# Autodesk Inventor assembly: Hatch design
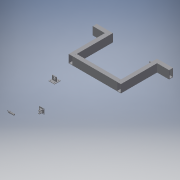
[picture p0: Inventor's stored thumbnail of the model, 180x180]
Saved by Autodesk Inventor 2018 (Build 220112000, 112)
## iProperties
Created: 2019-01-16
Part Number: Hatch design
Document SubType Name: Assembly
Designer: s-4008082
Author: s-4008082
## Documents named in this file (7)
- C:\Users\s-4008082\Downloads\hatch\Hatch design.iam
- C:\Users\s-4008082\Downloads\hatch\left arm.ipt
- C:\Users\s-4008082\Downloads\hatch\right arm.ipt
- C:\Users\s-4008082\Downloads\hatch\pneumatics back holder.ipt
- C:\Users\s-4008082\Downloads\hatch\pneumatics front holder.ipt
- C:\Users\s-4008082\Downloads\hatch\0070_011.iam
- C:\Users\s-4008082\Downloads\hatch\platform.ipt
## Components (9 placed, 6 different names)
1. left arm:1 — Mate:1, Mate:3, Mate:4, Mate:5, Flush:3, Mate:7, Flush:6, Flush:7
2. right arm:1 — Flush:4, Mate:6, Flush:5
3. pneumatics back holder:1 — Mate:3, Mate:5
4. pneumatics back holder:2
5. pneumatics front holder:1
6. pneumatics front holder:2 — Mate:1, Flush:1, Flush:2, Mate:2, Mate:4, Flush:3
7. 0070_011:1 [sub-assembly]
8. 0070_011:2 [sub-assembly] — Flush:1, Flush:2, Mate:2
9. platform:1 — Flush:4, Mate:6, Flush:5, Mate:7, Flush:6, Flush:7
## Relationships (14: Mate 7, Flush 7)
- Mate:1: left arm:1 ↔ pneumatics front holder:2
- Flush:1: pneumatics front holder:2 ↔ 0070_011:2
- Flush:2 (5.08 mm): pneumatics front holder:2 ↔ 0070_011:2
- Mate:2 (-7.62 mm): pneumatics front holder:2 ↔ 0070_011:2
- Mate:3: left arm:1 ↔ pneumatics back holder:1
- Mate:4: left arm:1 ↔ pneumatics front holder:2
- Mate:5: left arm:1 ↔ pneumatics back holder:1
- Flush:3: left arm:1 ↔ pneumatics front holder:2
- Flush:4: right arm:1 ↔ platform:1
- Mate:6: right arm:1 ↔ platform:1
- Flush:5: right arm:1 ↔ platform:1
- Mate:7: left arm:1 ↔ platform:1
- Flush:6: left arm:1 ↔ platform:1
- Flush:7: left arm:1 ↔ platform:1
